# Autodesk Inventor assembly: Obudowa_kapacz_dreczyciel
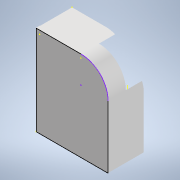
[picture p0: Inventor's stored thumbnail of the model, 180x180]
Saved by Autodesk Inventor 2022 (Build 260153000, 153)
## iProperties
Created: 2024-01-26
Part Number: Obudowa_kapacz_dreczyciel
Document SubType Name: Assembly
Designer: mateu
Author: mateu
## Documents named in this file (3)
- C:\Users\mateu\OneDrive\Dokumenty\Inventor\Obudowa_Komp_Wspom\Obudowa_kapacz_dreczyciel.iam
- C:\Users\mateu\OneDrive\Dokumenty\Inventor\Obudowa_Komp_Wspom\Dół.ipt
- C:\Users\mateu\OneDrive\Dokumenty\Inventor\Obudowa_Komp_Wspom\góra.ipt
## Components (2 placed, 2 different names)
1. Dół:1 — Mate:1
2. góra:1 — Mate:1
## Relationships (1: Mate 1)
- Mate:1: Dół:1 ↔ góra:1
